# Autodesk Inventor assembly: BottomRobot
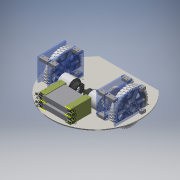
[picture p0: Inventor's stored thumbnail of the model, 180x180]
Saved by Autodesk Inventor 2019 (Build 230136000, 136)
## iProperties
Created: 2020-03-02
Part Number: BottomRobot
Document SubType Name: Assembly
Designer: james
Author: james
## Documents named in this file (6)
- F:\JimsRobot\FIRSTRobots\Design\TornadoPlatypus\BottomRobot.iam
- F:\JimsRobot\FIRSTRobots\Design\TornadoPlatypus\BottomPlate.ipt
- F:\JimsRobot\FIRSTRobots\Design\TornadoPlatypus\MotorLeft.iam
- F:\JimsRobot\FIRSTRobots\Design\TornadoPlatypus\MotorRight.iam
- F:\JimsRobot\FIRSTRobots\Design\Library\Jims\BatteryRail.ipt
- F:\JimsRobot\FIRSTRobots\Design\Library\RevRobotics\REV-31-1302.ipt
## Components (9 placed, 5 different names)
1. BottomPlate:1 — Mate:1, Mate:2, Mate:3, Mate:4, Mate:5, Mate:6, Mate:7, Mate:8, Mate:10, Mate:11, Mate:12
2. MotorLeft:1 [sub-assembly] — Mate:1, Mate:3, Mate:5
3. MotorRight:1 [sub-assembly] — Mate:2, Mate:4
4. BatteryRail:1 — Mate:6, Mate:7, Mate:8, Mate:9, Flush:1, Flush:2
5. BatteryRail:2 — Mate:10, Mate:11, Mate:12, Mate:13, Flush:3, Flush:4, Mate:14, Mate:15
6. BatteryRail:3 — Mate:9, Flush:1, Flush:2, Mate:16, Mate:17
7. BatteryRail:4 — Mate:13, Flush:3, Flush:4
8. REV-31-1302:1 — Mate:14, Mate:15
9. REV-31-1302:2 — Mate:16, Mate:17
## Relationships (21: Mate 17, Flush 4)
- Mate:1: BottomPlate:1 ↔ MotorLeft:1
- Mate:2: BottomPlate:1 ↔ MotorRight:1
- Mate:3: BottomPlate:1 ↔ MotorLeft:1
- Mate:4: BottomPlate:1 ↔ MotorRight:1
- Mate:5: BottomPlate:1 ↔ MotorLeft:1
- Mate:6: BottomPlate:1 ↔ BatteryRail:1
- Mate:7: BottomPlate:1 ↔ BatteryRail:1
- Mate:8: BottomPlate:1 ↔ BatteryRail:1
- Mate:9: BatteryRail:1 ↔ BatteryRail:3
- Flush:1: BatteryRail:1 ↔ BatteryRail:3
- Flush:2: BatteryRail:1 ↔ BatteryRail:3
- Mate:10: BottomPlate:1 ↔ BatteryRail:2
- Mate:11: BottomPlate:1 ↔ BatteryRail:2
- Mate:12: BottomPlate:1 ↔ BatteryRail:2
- Mate:13: BatteryRail:2 ↔ BatteryRail:4
- Flush:3: BatteryRail:2 ↔ BatteryRail:4
- Flush:4: BatteryRail:2 ↔ BatteryRail:4
- Mate:14: BatteryRail:2 ↔ REV-31-1302:1
- Mate:15: BatteryRail:2 ↔ REV-31-1302:1
- Mate:16: BatteryRail:3 ↔ REV-31-1302:2
- Mate:17: BatteryRail:3 ↔ REV-31-1302:2
